# Autodesk Inventor assembly: Donna
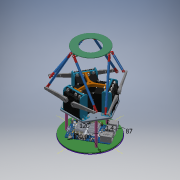
[picture p0: Inventor's stored thumbnail of the model, 180x180]
Saved by Autodesk Inventor 2018.2 (Build 222227000, 227)
## iProperties
Created: 2018-02-19
Part Number: Donna
Material: Generisch
Document SubType Name: Assembly
Designer: JochenAlt
Author: JochenAlt
## Documents named in this file (6)
- D:\Projects\Donna\CAD\Donna.iam
- D:\Projects\Donna\CAD\Base-Plate.ipt
- D:\Projects\Donna\CAD\Stewart-Platform-Inside.iam
- D:\Projects\Donna\CAD\Base-Stewart-Connector.ipt
- D:\Projects\Donna\CAD\ODroid C2\ODroid C2.iam
- D:\Projects\Donna\CAD\Teensy 3.5-3.6\Teensy.iam
## Components (7 placed, 5 different names)
1. Base-Plate:1 — Passend:1, Passend:2, Passend:3, Passend:4, Passend:5, Passend:6, Winkel:1, Passend:10, Winkel:3
2. Stewart Platform Inside:1 [sub-assembly] — Passend:7, Passend:8, Passend:9, Winkel:2
3. Base-Stewart-Connector:1 — Passend:2, Passend:6, Passend:9
4. Base-Stewart-Connector:2 — Passend:3, Passend:4, Passend:8
5. Base-Stewart-Connector:3 — Passend:1, Passend:5, Passend:7
6. ODroid C2:1 [sub-assembly] — Winkel:1, Winkel:2, Passend:10, Winkel:4
7. Teensy:1 [sub-assembly] — Winkel:3, Winkel:4
## Relationships (14: Mate 10, Angle 4)
- Passend:1 [Mate]: Base-Plate:1 ↔ Base-Stewart-Connector:3
- Passend:2 [Mate]: Base-Plate:1 ↔ Base-Stewart-Connector:1
- Passend:3 [Mate]: Base-Plate:1 ↔ Base-Stewart-Connector:2
- Passend:4 [Mate]: Base-Plate:1 ↔ Base-Stewart-Connector:2
- Passend:5 [Mate]: Base-Plate:1 ↔ Base-Stewart-Connector:3
- Passend:6 [Mate]: Base-Plate:1 ↔ Base-Stewart-Connector:1
- Passend:7 [Mate]: Stewart Platform Inside:1 ↔ Base-Stewart-Connector:3
- Passend:8 [Mate]: Stewart Platform Inside:1 ↔ Base-Stewart-Connector:2
- Passend:9 [Mate]: Stewart Platform Inside:1 ↔ Base-Stewart-Connector:1
- Winkel:1 [Angle] (180 deg): Base-Plate:1 ↔ ODroid C2:1
- Winkel:2 [Angle] (0 deg): Stewart Platform Inside:1 ↔ ODroid C2:1
- Passend:10 [Mate] (5 mm): Base-Plate:1 ↔ ODroid C2:1
- Winkel:3 [Angle] (0 deg): Base-Plate:1 ↔ Teensy:1
- Winkel:4 [Angle] (180 deg): ODroid C2:1 ↔ Teensy:1
